# Autodesk Inventor assembly: base
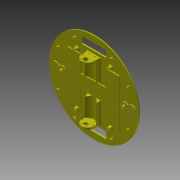
[picture p0: Inventor's stored thumbnail of the model, 180x180]
Saved by Autodesk Inventor 2015 (Build 190159000, 159)
## iProperties
Created: 2015-03-17
Part Number: base
Document SubType Name: Assembly
Designer: david_000
Author: david_000
## Documents named in this file (5)
- C:\Users\david_000\Desktop\minibot-code\mechanics\base.iam
- C:\Users\david_000\Desktop\minibot-code\mechanics\base_1.ipt
- C:\Users\david_000\Desktop\minibot-code\mechanics\base_2.ipt
- C:\Users\david_000\Desktop\minibot-code\mechanics\base_3.ipt
- C:\Users\david_000\Desktop\minibot-code\mechanics\pie.ipt
## Components (7 placed, 4 different names)
1. base_3:1 — Coincidencia:7, Coincidencia:8, Coincidencia:9, Coincidencia:10, Coincidencia:11, Coincidencia:12, Coincidencia:13, Coincidencia:14, Coincidencia:15
2. base_1:3 — Coincidencia:7, Coincidencia:8, Coincidencia:9, Nivelación:1, Nivelación:2, Coincidencia:16, Coincidencia:17, Coincidencia:18
3. base_1:4 — Coincidencia:10, Coincidencia:11, Nivelación:1, Coincidencia:19, Coincidencia:20, Coincidencia:21
4. base_2:3 — Nivelación:3, Coincidencia:14, Coincidencia:15
5. base_2:4 — Coincidencia:12, Coincidencia:13, Nivelación:2, Nivelación:3
6. pie:1 — Coincidencia:16, Coincidencia:17, Coincidencia:18
7. pie:2 — Coincidencia:19, Coincidencia:20, Coincidencia:21
## Relationships (18: Mate 15, Flush 3)
- Coincidencia:7 [Mate]: base_3:1 ↔ base_1:3
- Coincidencia:8 [Mate]: base_3:1 ↔ base_1:3
- Coincidencia:9 [Mate]: base_3:1 ↔ base_1:3
- Coincidencia:10 [Mate]: base_3:1 ↔ base_1:4
- Coincidencia:11 [Mate]: base_3:1 ↔ base_1:4
- Nivelación:1 [Flush]: base_1:3 ↔ base_1:4
- Coincidencia:12 [Mate]: base_3:1 ↔ base_2:4
- Coincidencia:13 [Mate]: base_3:1 ↔ base_2:4
- Nivelación:2 [Flush]: base_1:3 ↔ base_2:4
- Nivelación:3 [Flush]: base_2:3 ↔ base_2:4
- Coincidencia:14 [Mate]: base_3:1 ↔ base_2:3
- Coincidencia:15 [Mate]: base_3:1 ↔ base_2:3
- Coincidencia:16 [Mate]: base_1:3 ↔ pie:1
- Coincidencia:17 [Mate]: base_1:3 ↔ pie:1
- Coincidencia:18 [Mate]: base_1:3 ↔ pie:1
- Coincidencia:19 [Mate]: base_1:4 ↔ pie:2
- Coincidencia:20 [Mate]: base_1:4 ↔ pie:2
- Coincidencia:21 [Mate]: base_1:4 ↔ pie:2
